# Autodesk Inventor assembly: stepper_motor
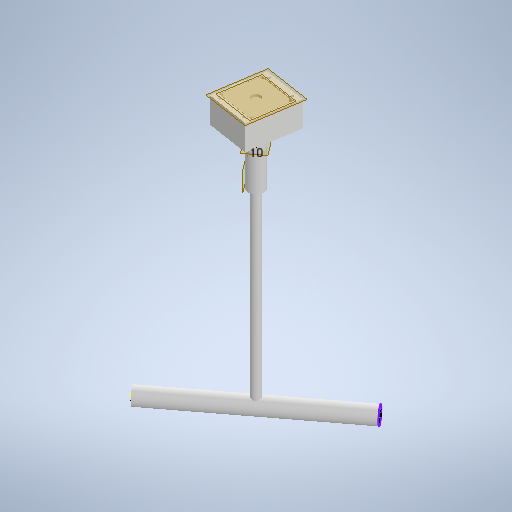
[picture p0: Inventor's stored thumbnail of the model, 512x512]
Saved by Autodesk Inventor 2025.2 (Build 292293000, 293)
## iProperties
Created: 2024-11-23
Part Number: stepper_motor
Document SubType Name: Assembly
Designer: dell
Author: dell
## Documents named in this file (4)
- D:\兵庫県立大\creap\Tonbo.iam
- D:\兵庫県立大\creap\joint.ipt
- D:\兵庫県立大\creap\Tonbo.ipt
- D:\兵庫県立大\creap\motor_case.iam
## Components (3 placed, 3 different names)
1. joint:1 — リジッド:2, 回転:4
2. Tonbo:1 — リジッド:2
3. motor_case:1 [sub-assembly] — 回転:4
## Relationships (2: WeldJoint 1, RevoluteJoint 1)
- リジッド:2 [WeldJoint]: joint:1 ↔ Tonbo:1
- 回転:4 [RevoluteJoint]: joint:1 ↔ motor_case:1
